# Autodesk Inventor assembly: brush end effector
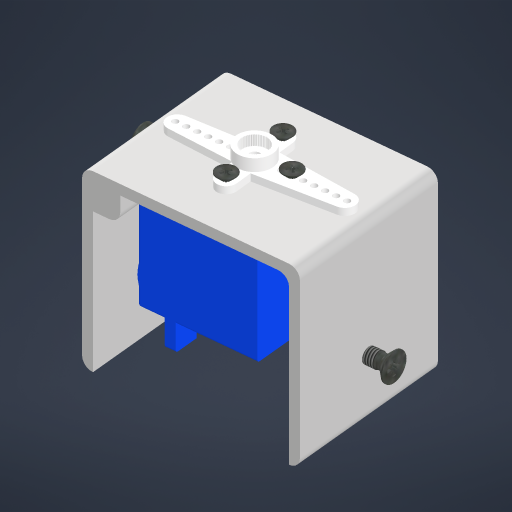
[picture p0: Inventor's stored thumbnail of the model, 512x512]
Saved by Autodesk Inventor 2024.2 (Build 282272000, 272)
## iProperties
Created: 2024-03-20
Part Number: brush end effector
Document SubType Name: Assembly
Designer: seifs
Author: seifs
## Documents named in this file (9)
- C:\Users\seifs\Downloads\Right Side Assembly\brush end effector_2.iam
- C:\Users\seifs\Downloads\Right Side Assembly\Servo Motor SG90.ipt
- C:\Users\seifs\Downloads\Right Side Assembly\SG90 - Micro Servo 9g - Tower Pro.4.ipt
- C:\Users\seifs\Downloads\Right Side Assembly\Pan and tilt final part.ipt
- C:\Users\seifs\OneDrive\Documents\Inventor\Content Center Files\R2024\en-US\ISO 7046-1 Z(1)\ISO 7046-1 - M3 x 12_ - 4.8 - Z - ISO.ipt
- C:\Users\seifs\OneDrive\Documents\Inventor\Content Center Files\R2024\en-US\ISO 4036(2)\ISO 4036 - M3(2).ipt
- C:\Users\seifs\OneDrive\Documents\Inventor\Content Center Files\R2024\en-US\ISO 7046-1 Z(1)\ISO 7046-1 - M3 x 16_ - 4.8 - Z - ISO.ipt
- C:\Users\seifs\OneDrive\Documents\Inventor\Content Center Files\R2024\en-US\ISO 7046-1 Z(1)\ISO 7046-1 - M2 x 8_ - 4.8 - Z - ISO.ipt
- C:\Users\seifs\OneDrive\Documents\Inventor\Content Center Files\R2024\en-US\ISO 4036(2)\ISO 4036 - M2(2).ipt
## Components (13 placed, 8 different names)
1. SG90 - Micro Servo 9g - Tower Pro.4:1 — Insert:4, Mate:1, Mate:2, Insert:20, Insert:21, Insert:22
2. Servo Motor SG90:2 — Insert:5, Mate:3, Insert:19
3. Pan and tilt final part:1 — Insert:4, Insert:5, Mate:1, Mate:2, Mate:3, Insert:13, Insert:18, Insert:23, Insert:24, Insert:25
4. ISO 7046-1 Z M3 x 12 - 4.8 - Z:1
5. ISO 4036 M3:1 — Insert:13
6. ISO 7046-1 Z M3 x 16 - 4.8 - Z:1 — Insert:18
7. ISO 4036 M3:4 — Insert:19
8. ISO 7046-1 Z M2 x 8 - 4.8 - Z:1 — Insert:20
9. ISO 7046-1 Z M2 x 8 - 4.8 - Z:2 — Insert:21
10. ISO 7046-1 Z M2 x 8 - 4.8 - Z:3 — Insert:22
11. ISO 4036 M2:1 — Insert:23
12. ISO 4036 M2:2 — Insert:25
13. ISO 4036 M2:3 — Insert:24
## Relationships (14: Insert 11, Mate 3)
- Insert:4: SG90 - Micro Servo 9g - Tower Pro.4:1 ↔ Pan and tilt final part:1
- Insert:5: Servo Motor SG90:2 ↔ Pan and tilt final part:1
- Mate:1: SG90 - Micro Servo 9g - Tower Pro.4:1 ↔ Pan and tilt final part:1
- Mate:2: SG90 - Micro Servo 9g - Tower Pro.4:1 ↔ Pan and tilt final part:1
- Mate:3: Servo Motor SG90:2 ↔ Pan and tilt final part:1
- Insert:13: Pan and tilt final part:1 ↔ ISO 4036 M3:1
- Insert:18: Pan and tilt final part:1 ↔ ISO 7046-1 Z M3 x 16 - 4.8 - Z:1
- Insert:19: Servo Motor SG90:2 ↔ ISO 4036 M3:4
- Insert:20: SG90 - Micro Servo 9g - Tower Pro.4:1 ↔ ISO 7046-1 Z M2 x 8 - 4.8 - Z:1
- Insert:21: SG90 - Micro Servo 9g - Tower Pro.4:1 ↔ ISO 7046-1 Z M2 x 8 - 4.8 - Z:2
- Insert:22: SG90 - Micro Servo 9g - Tower Pro.4:1 ↔ ISO 7046-1 Z M2 x 8 - 4.8 - Z:3
- Insert:23: Pan and tilt final part:1 ↔ ISO 4036 M2:1
- Insert:24: Pan and tilt final part:1 ↔ ISO 4036 M2:3
- Insert:25: Pan and tilt final part:1 ↔ ISO 4036 M2:2
